# Autodesk Inventor assembly: Сборка
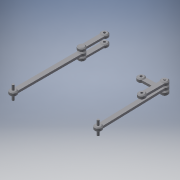
[picture p0: Inventor's stored thumbnail of the model, 180x180]
Saved by Autodesk Inventor 2018 (Build 220112000, 112)
## iProperties
Created: 2018-11-12
Part Number: Сборка
Material: Типовые
Document SubType Name: Assembly
Designer: Lev
Author: Lev
## Documents named in this file (5)
- C:\Users\Lev\Documents\Прикмех\Сборка.iam
- C:\Users\Lev\Documents\Прикмех\Деталь1.ipt
- C:\Users\Lev\Documents\Прикмех\Деталь2.ipt
- C:\Users\Lev\Documents\Прикмех\Деталь2_б.ipt
- C:\Users\Lev\Documents\Прикмех\Палец.ipt
## Components (8 placed, 4 different names)
1. Деталь1:1 — Совмещение:1, С поворотом:1, С поворотом:4
2. Деталь2:1 — Совмещение:1, С поворотом:1
3. Деталь2_б:1 — С поворотом:7
4. Палец:1 — С поворотом:3
5. Деталь1:2 — С поворотом:3, С поворотом:5, С поворотом:6, С поворотом:7
6. Палец:4 — С поворотом:5
7. Деталь2_б:2 — С поворотом:6
8. Палец:5 — С поворотом:4
## Relationships (7: RevoluteJoint 6, Mate 1)
- Совмещение:1 [Mate]: Деталь1:1 ↔ Деталь2:1
- С поворотом:1 [RevoluteJoint]: Деталь1:1 ↔ Деталь2:1
- С поворотом:3 [RevoluteJoint]: Палец:1 ↔ Деталь1:2
- С поворотом:4 [RevoluteJoint]: Деталь1:1 ↔ Палец:5
- С поворотом:5 [RevoluteJoint]: Деталь1:2 ↔ Палец:4
- С поворотом:6 [RevoluteJoint]: Деталь1:2 ↔ Деталь2_б:2
- С поворотом:7 [RevoluteJoint]: Деталь2_б:1 ↔ Деталь1:2
